# Autodesk Inventor assembly: AssemblyV1
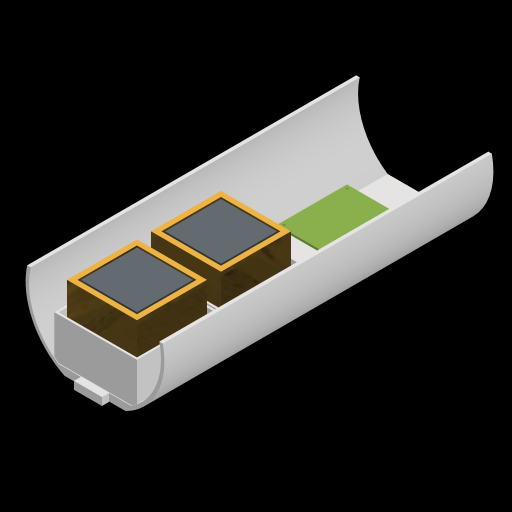
[picture p0: Inventor's stored thumbnail of the model, 512x512]
Saved by Autodesk Inventor 2024 (Build 280153000, 153)
## iProperties
Created: 2026-04-10
Part Number: AssemblyV1
Document SubType Name: Assembly
Designer: Tanner
Author: Tanner
## Documents named in this file (12)
- C:\Users\Tanner\Documents\Inventor\Proton Magnetometer V2\AssemblyV1.iam
- C:\Users\Tanner\Documents\Inventor\Proton Magnetometer V2\FrontTubeV1.ipt
- C:\Users\Tanner\Documents\Inventor\Proton Magnetometer V2\FrontCapV1.ipt
- C:\Users\Tanner\Documents\Inventor\Proton Magnetometer V2\BackTubeV1.ipt
- C:\Users\Tanner\Documents\Inventor\Proton Magnetometer V2\BackCapV2.ipt
- C:\Users\Tanner\Documents\Inventor\Proton Magnetometer V2\OringV2.ipt
- C:\Users\Tanner\Documents\Inventor\Proton Magnetometer V2\InsertV1.ipt
- C:\Users\Tanner\Documents\Inventor\Proton Magnetometer V2\BackInsertV1.ipt
- C:\Users\Tanner\Documents\Inventor\Proton Magnetometer V2\BottleV1.ipt
- C:\Users\Tanner\Documents\Inventor\Proton Magnetometer V2\CoilV1.ipt
- C:\Users\Tanner\Documents\Inventor\Proton Magnetometer V2\PCBV1.ipt
- C:\Users\Tanner\Documents\Inventor\Proton Magnetometer V2\FrontBumper.ipt
## Components (13 placed, 11 different names)
1. FrontTubeV1:1 — Flush:1, Mate:1, Mate:2, Angle:1, Flush:5
2. FrontCapV1:1 — Flush:1, Flush:4
3. BackTubeV1:1 — Mate:1, Mate:2, Angle:1, Flush:2, Mate:3, Flush:3
4. BackCapV2:1 — Flush:2, Flush:4
5. OringV2:1 — Mate:3, Flush:3
6. InsertV1:1 — Flush:5, Flush:6, Mate:5, Mate:6, Mate:13, Mate:14, Flush:7, Flush:9, Flush:10
7. BackInsertV1:1 — Flush:6, Mate:4, Mate:7, Mate:16, Flush:8, Mate:17
8. BottleV1:1 — Mate:9, Mate:10, Mate:13
9. BottleV1:2 — Mate:11, Mate:12, Mate:14
10. CoilV1:1 — Mate:4, Mate:5, Mate:8, Mate:9, Mate:10, Flush:7
11. CoilV1:2 — Mate:6, Mate:7, Mate:8, Mate:11, Mate:12
12. PCBV1:1 — Mate:16, Flush:8, Mate:17
13. FrontBumper:1 — Flush:9, Flush:10
## Relationships (27: Mate 16, Flush 10, Angle 1)
- Flush:1: FrontTubeV1:1 ↔ FrontCapV1:1
- Mate:1: FrontTubeV1:1 ↔ BackTubeV1:1
- Mate:2: FrontTubeV1:1 ↔ BackTubeV1:1
- Angle:1 (0 deg): FrontTubeV1:1 ↔ BackTubeV1:1
- Flush:2: BackTubeV1:1 ↔ BackCapV2:1
- Mate:3: BackTubeV1:1 ↔ OringV2:1
- Flush:3: BackTubeV1:1 ↔ OringV2:1
- Flush:4: FrontCapV1:1 ↔ BackCapV2:1
- Flush:5: FrontTubeV1:1 ↔ InsertV1:1
- Flush:6: InsertV1:1 ↔ BackInsertV1:1
- Mate:4 (5 mm): BackInsertV1:1 ↔ CoilV1:1
- Mate:5: InsertV1:1 ↔ CoilV1:1
- Mate:6: InsertV1:1 ↔ CoilV1:2
- Mate:7 (5 mm): BackInsertV1:1 ↔ CoilV1:2
- Mate:8 (20 mm): CoilV1:1 ↔ CoilV1:2
- Mate:9 (2.5 mm): BottleV1:1 ↔ CoilV1:1
- Mate:10 (2.5 mm): BottleV1:1 ↔ CoilV1:1
- Mate:11 (2.5 mm): BottleV1:2 ↔ CoilV1:2
- Mate:12 (2.5 mm): BottleV1:2 ↔ CoilV1:2
- Mate:13 (5 mm): InsertV1:1 ↔ BottleV1:1
- Mate:14 (5 mm): InsertV1:1 ↔ BottleV1:2
- Flush:7 (10 mm): InsertV1:1 ↔ CoilV1:1
- Mate:16: BackInsertV1:1 ↔ PCBV1:1
- Flush:8 (60 mm): BackInsertV1:1 ↔ PCBV1:1
- Flush:9: InsertV1:1 ↔ FrontBumper:1
- Flush:10: InsertV1:1 ↔ FrontBumper:1
- Mate:17 (15 mm): BackInsertV1:1 ↔ PCBV1:1
